# Autodesk Inventor assembly: frameAssembly
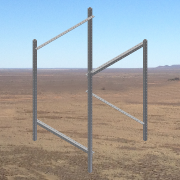
[picture p0: Inventor's stored thumbnail of the model, 180x180]
Saved by Autodesk Inventor 2014 SP1 (Build 180222100, 222)
## iProperties
Created: 2014-05-23
Part Number: frameAssembly
Document SubType Name: Assembly
Designer: Dave
Author: Dave
## Documents named in this file (3)
- C:\Users\Dave\Desktop\hera-cad\Node\frameAssembly.iam
- C:\Users\Dave\Desktop\hera-cad\Node\frame_uni_vert.ipt
- C:\Users\Dave\Desktop\hera-cad\Node\frame_angle_horiz.ipt
## Components (8 placed, 2 different names)
1. frame_angle_horiz:1 — Insert:1
2. frame_angle_horiz:2 — Insert:2
3. frame_angle_horiz:3 — Insert:4
4. frame_angle_horiz:4 — Insert:3
5. frame_uni_vert:1 — Insert:4
6. frame_uni_vert:2
7. frame_uni_vert:3 — Insert:2, Insert:3
8. frame_uni_vert:4 — Insert:1
## Component patterns: (4 elements, first: frame_uni_vert:1)
## Relationships (4: Insert 4)
- Insert:1: frame_angle_horiz:1 ↔ frame_uni_vert:4
- Insert:2: frame_angle_horiz:2 ↔ frame_uni_vert:3
- Insert:3: frame_angle_horiz:4 ↔ frame_uni_vert:3
- Insert:4: frame_angle_horiz:3 ↔ frame_uni_vert:1
